# Autodesk Inventor assembly: robot
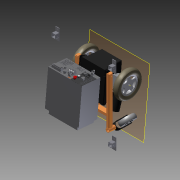
[picture p0: Inventor's stored thumbnail of the model, 180x180]
Saved by Autodesk Inventor 2012 (Build 160160000, 160)
## iProperties
Created: 2012-03-08
Part Number: robot
Document SubType Name: Assembly
Designer: esv
Author: esv
## Documents named in this file (4)
- C:\Users\esv\masters\CAD\robot.iam
- C:\Users\esv\masters\CAD\Frame\frame bracket.ipt
- C:\Users\esv\masters\CAD\Invacare\invacare assy.iam
- C:\Users\esv\Documents\Inventor\IRC5_Compact.ipt
## Components (6 placed, 3 different names)
1. frame bracket:1 — Mate:3, Flush:4, Angle:1, Flush:5
2. frame bracket:2 — Mate:5, Flush:6, Flush:7
3. frame bracket:3 — Mate:2, Flush:4, Flush:6
4. frame bracket:4 — Flush:5, Mate:4, Flush:7
5. invacare assy:1 [sub-assembly] — Mate:1, Flush:1, Flush:3, Mate:2, Mate:3, Angle:1, Mate:4, Mate:5
6. IRC5_Compact:1 — Mate:1, Flush:1, Flush:2
## Relationships (13: Flush 7, Mate 5, Angle 1)
- Mate:1 (127 mm): invacare assy:1 ↔ IRC5_Compact:1
- Flush:1: invacare assy:1 ↔ IRC5_Compact:1
- Flush:2 (-225 mm): IRC5_Compact:1
- Flush:3: invacare assy:1
- Mate:2: frame bracket:3 ↔ invacare assy:1
- Mate:3: frame bracket:1 ↔ invacare assy:1
- Flush:4: frame bracket:1 ↔ frame bracket:3
- Angle:1 (0 deg): frame bracket:1 ↔ invacare assy:1
- Flush:5: frame bracket:1 ↔ frame bracket:4
- Mate:4: frame bracket:4 ↔ invacare assy:1
- Mate:5: frame bracket:2 ↔ invacare assy:1
- Flush:6: frame bracket:2 ↔ frame bracket:3
- Flush:7: frame bracket:2 ↔ frame bracket:4
